# Autodesk Inventor assembly: Shoulder base
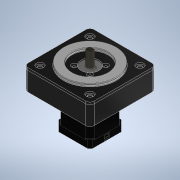
[picture p0: Inventor's stored thumbnail of the model, 180x180]
Saved by Autodesk Inventor 2022 (Build 260153000, 153)
## iProperties
Created: 2022-03-02
Part Number: Shoulder base
Document SubType Name: Assembly
Designer: JK
Author: JK
## Documents named in this file (6)
- C:\Users\JK\Documents\Inventor\ScaraNema\SCARA-3DP\Parts\Shoulder\Shoulder base.iam
- C:\Users\JK\Documents\Inventor\ScaraNema\SCARA-3DP\Parts\Shoulder\17HS15-1684S-PG5.ipt
- C:\Users\JK\Documents\Inventor\ScaraNema\SCARA-3DP\Parts\Shoulder\Motor Support Plate.ipt
- C:\Users\JK\Documents\Inventor\ScaraNema\SCARA-3DP\Parts\Shoulder\Base.ipt
- C:\Users\JK\Documents\Inventor\ScaraNema\SCARA-3DP\Parts\Shoulder\Needle roller bearing\5909K79_1 mm Thick Washer for 45 mm Shaft Diameter Needle-Roller Thrust Bearing.ipt
- C:\Users\JK\Documents\Inventor\ScaraNema\SCARA-3DP\Parts\Shoulder\Needle roller bearing\5909K19_Needle-Roller Thrust Bearing.ipt
## Components (6 placed, 5 different names)
1. 17HS15-1684S-PG5:1 — Coincidencia:1, Coincidencia:2, Coincidencia:3, Coincidencia:4, Coincidencia:9, Coincidencia:10
2. Motor Support Plate:1 — Coincidencia:1, Coincidencia:2, Coincidencia:3, Coincidencia:5, Coincidencia:6, Coincidencia:7, Coincidencia:8
3. Base:1 — Coincidencia:4, Coincidencia:5, Coincidencia:6
4. 5909K79_1 mm Thick Washer for 45 mm Shaft Diameter Needle-Roller Thrust Bearing:1 — Coincidencia:7, Coincidencia:8, Tangente:1
5. 5909K19_Needle-Roller Thrust Bearing:1 — Coincidencia:9, Tangente:1, Tangente:2
6. 5909K79_1 mm Thick Washer for 45 mm Shaft Diameter Needle-Roller Thrust Bearing:2 — Coincidencia:10, Tangente:2
## Relationships (12: Mate 10, Tangent 2)
- Coincidencia:1 [Mate]: 17HS15-1684S-PG5:1 ↔ Motor Support Plate:1
- Coincidencia:2 [Mate]: 17HS15-1684S-PG5:1 ↔ Motor Support Plate:1
- Coincidencia:3 [Mate]: 17HS15-1684S-PG5:1 ↔ Motor Support Plate:1
- Coincidencia:4 [Mate]: 17HS15-1684S-PG5:1 ↔ Base:1
- Coincidencia:5 [Mate]: Motor Support Plate:1 ↔ Base:1
- Coincidencia:6 [Mate]: Motor Support Plate:1 ↔ Base:1
- Coincidencia:7 [Mate]: Motor Support Plate:1 ↔ 5909K79_1 mm Thick Washer for 45 mm Shaft Diameter Needle-Roller Thrust Bearing:1
- Coincidencia:8 [Mate]: Motor Support Plate:1 ↔ 5909K79_1 mm Thick Washer for 45 mm Shaft Diameter Needle-Roller Thrust Bearing:1
- Coincidencia:9 [Mate]: 17HS15-1684S-PG5:1 ↔ 5909K19_Needle-Roller Thrust Bearing:1
- Tangente:1: 5909K79_1 mm Thick Washer for 45 mm Shaft Diameter Needle-Roller Thrust Bearing:1 ↔ 5909K19_Needle-Roller Thrust Bearing:1
- Coincidencia:10 [Mate]: 17HS15-1684S-PG5:1 ↔ 5909K79_1 mm Thick Washer for 45 mm Shaft Diameter Needle-Roller Thrust Bearing:2
- Tangente:2: 5909K19_Needle-Roller Thrust Bearing:1 ↔ 5909K79_1 mm Thick Washer for 45 mm Shaft Diameter Needle-Roller Thrust Bearing:2
